(part 1 of 3)
# Autodesk Inventor assembly: Final
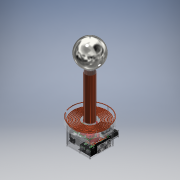
[picture p0: Inventor's stored thumbnail of the model, 180x180]
Saved by Autodesk Inventor 2019 (Build 230136000, 136)
## iProperties
Created: 2018-05-15
Part Number: Final
Document SubType Name: Assembly
Designer: Phil Erle
Author: Phil Erle
## Documents named in this file (78)
- C:\Users\Erle\Desktop\CAD\Final.iam
- C:\Users\Erle\Desktop\CAD\bottom.ipt
- C:\Users\Erle\Desktop\CAD\Elektronik_Gehäuse.ipt
- C:\Users\Erle\Desktop\CAD\Heatsink.ipt
- C:\Users\Erle\Desktop\CAD\EndStück_Caps.ipt
- C:\Users\Erle\Desktop\CAD\SeitenUntenVorne.ipt
- C:\Users\Erle\Desktop\CAD\SeitenUntenHinten.ipt
- C:\Users\Erle\Desktop\CAD\Cap.ipt
- C:\Users\Erle\Desktop\CAD\mid.ipt
- C:\Users\Erle\Desktop\CAD\MidStück_Caps.ipt
- C:\Users\Erle\Desktop\CAD\LogicHolder.ipt
- C:\Users\Erle\Desktop\CAD\NtHolder.ipt
- C:\Users\Erle\Desktop\CAD\SeitenUnten.ipt
- C:\Users\Erle\Desktop\CAD\ToslinkHalter.ipt
- C:\Users\Erle\Desktop\CAD\IGBT_Platine.ipt
- C:\Users\Erle\Desktop\CAD\GT175DA120U.ipt
- C:\Users\Erle\Desktop\CAD\Abstandshalter_12mm_M4.ipt
- C:\Users\Erle\Desktop\CAD\Normteile\Unterlegscheiben\din125-1-a_4_3-140_hv.ipt
- C:\Users\Erle\Desktop\CAD\CU6.ipt
- C:\Users\Erle\Desktop\CAD\CU5.ipt
- C:\Users\Erle\Desktop\CAD\Snubber.ipt
- C:\Users\Erle\Desktop\CAD\CU7.ipt
- C:\Users\Erle\Desktop\CAD\CU8.ipt
- C:\Users\Erle\Desktop\CAD\Normteile\Schrauben\M4\Zylinderkopf\din_en_iso_4762_m4x6.ipt
- C:\Users\Erle\Desktop\CAD\Normteile\Muttern\mutter_din934_m4-10.ipt
- C:\Users\Erle\Desktop\CAD\Cap_Platine.ipt
- C:\Users\Erle\Desktop\CAD\Main.ipt
- C:\Users\Erle\Desktop\CAD\SeitenOben.ipt
- C:\Users\Erle\Desktop\CAD\Abstandshalter_10mm.ipt
- C:\Users\Erle\Desktop\CAD\M5 Gewindestange.ipt
- C:\Users\Erle\Desktop\CAD\Normteile\Muttern\mutter_din934_m5-6.ipt
- C:\Users\Erle\Desktop\CAD\PlexiHalter1.ipt
- C:\Users\Erle\Desktop\CAD\PlexiHalter2.ipt
- C:\Users\Erle\Desktop\CAD\Primary.ipt
- C:\Users\Erle\Desktop\CAD\Seconday_End_Bottom.ipt
- C:\Users\Erle\Desktop\CAD\Seconday_End_Top.ipt
- C:\Users\Erle\Desktop\CAD\Normteile\Muttern\din1587-m5x0_8ricu3.ipt
- C:\Users\Erle\Desktop\CAD\Normteile\Muttern\mutter_din934_m6-6.ipt
- C:\Users\Erle\Desktop\CAD\Normteile\Muttern\din1587-m6x1ricu3.ipt
- C:\Users\Erle\Desktop\CAD\Secondary.ipt
- C:\Users\Erle\Desktop\CAD\Coil.ipt
- C:\Users\Erle\Desktop\CAD\M6 Gewindestange.ipt
- C:\Users\Erle\Desktop\CAD\TopLoad.ipt
- C:\Users\Erle\Desktop\CAD\primary_holder.ipt
- C:\Users\Erle\Desktop\CAD\Normteile\Schrauben\M3\din_en_iso_4762_m3x8.ipt
- C:\Users\Erle\Desktop\CAD\Normteile\Schrauben\M4\Zylinderkopf\din_en_iso_4762_m4x12.ipt
- C:\Users\Erle\Desktop\CAD\Normteile\Schrauben\M3\din_en_iso_4762_m3x10.ipt
- C:\Users\Erle\Desktop\CAD\Normteile\Muttern\mutter_din934_m3-6.ipt
- C:\Users\Erle\Desktop\CAD\Normteile\Schrauben\M3\din_en_iso_7991_m3x16.ipt
- C:\Users\Erle\Desktop\CAD\top.ipt
- C:\Users\Erle\Desktop\CAD\Strike_Rail.ipt
- C:\Users\Erle\Desktop\CAD\Power_Supply_S_90_18.ipt
- C:\Users\Erle\Desktop\CAD\M5 Gewindestange_Cap.ipt
- C:\Users\Erle\Desktop\CAD\Cu_Cap.ipt
- C:\Users\Erle\Desktop\CAD\Normteile\Unterlegscheiben\din125-1-a_5_3-140_hv.ipt
- C:\Users\Erle\Desktop\CAD\Platine_Gleichrichter.ipt
- C:\Users\Erle\Desktop\CAD\M6 Gewindestange_Unten.ipt
- C:\Users\Erle\Desktop\CAD\Gleichrichter.ipt
- C:\Users\Erle\Desktop\CAD\Netzfilter.ipt
- C:\Users\Erle\Desktop\CAD\Schalter.ipt
- C:\Users\Erle\Desktop\CAD\Netzstecker.ipt
- C:\Users\Erle\Desktop\CAD\Cap_CU_Oben.ipt
- C:\Users\Erle\Desktop\CAD\Normteile\Schrauben\M6\din_en_iso_4762_m6x10.ipt
- C:\Users\Erle\Desktop\CAD\Normteile\Schrauben\M5\din_en_iso_4762_m5x10.ipt
- C:\Users\Erle\Desktop\CAD\Normteile\Schrauben\M3\din_en_iso_4762_m3x25.ipt
- C:\Users\Erle\Desktop\CAD\Normteile\Schrauben\M3\din_en_iso_4762_m3x6.ipt
- C:\Users\Erle\Desktop\CAD\PrimaryCoil.ipt
- C:\Users\Erle\Desktop\CAD\Lüfter.ipt
- C:\Users\Erle\Desktop\CAD\Abstandshalter_5mm.ipt
- C:\Users\Erle\Desktop\CAD\GDT.ipt
- C:\Users\Erle\Desktop\CAD\Normteile\Schrauben\M3\din_en_iso_7991_m3x10.ipt
- C:\Users\Erle\Desktop\CAD\Normteile\Schrauben\M4\Zylinderkopf\din_en_iso_7991_m4x35.ipt
- C:\Users\Erle\Desktop\CAD\Rändelmutter.ipt
- C:\Users\Erle\Desktop\CAD\Lüftergitter.ipt
- C:\Users\Erle\Desktop\CAD\Normteile\Schrauben\M4\Zylinderkopf\din_en_iso_4762_m4x16.ipt
- C:\Users\Erle\Desktop\CAD\Normteile\Unterlegscheiben\din125-1-a_3_2-140_hv.ipt
- C:\Users\Erle\Desktop\CAD\CT.ipt
- C:\Users\Erle\Desktop\CAD\CT_Holder.ipt
## Components (478 placed, 77 different names)
1. bottom:1 — Flush:1, Flush:2, Mate:1, Mate:2, Mate:3, Mate:4, Mate:8, Mate:9, Mate:10, Mate:27, Mate:28, Mate:29, Mate:33, Mate:36, Mate:37, Mate:38, Mate:39, Mate:40, Mate:41, Mate:273, Mate:274, Mate:275, Flush:9, Flush:10, Flush:11, Flush:12, Mate:312, Mate:313, Mate:314, Mate:315, Mate:480, Mate:487, Mate:574, Mate:575, Mate:576, Mate:577, Mate:666, Mate:667, Mate:668, Mate:669, Mate:670, Mate:671, Mate:672, Mate:673, Mate:917, Mate:934, Mate:1121, Mate:1127, Mate:1132, Mate:1135
2. Elektronik_Gehäuse:1 — Mate:31, Mate:32, Mate:1106
3. Heatsink:1 — Mate:8, Mate:9, Mate:10, Mate:45, Mate:46, Mate:47, Mate:48, Mate:49, Mate:50, Mate:51, Mate:52, Mate:53, Mate:54, Mate:55, Mate:56, Mate:565, Mate:566, Angle:6, Mate:658, Mate:661, Mate:664, Mate:665, Mate:887, Mate:888, Mate:889, Mate:890, Mate:891, Mate:892, Mate:893, Mate:894, Mate:895, Mate:896, Mate:897, Mate:898
4. EndStück_Caps:1 — Mate:18, Mate:19, Mate:20, Mate:22, Mate:499, Mate:500, Mate:501, Mate:502, Flush:476, Flush:477, Flush:478, Flush:479, Mate:503, Mate:504, Mate:505, Mate:506
5. EndStück_Caps:2 — Mate:11, Mate:12, Mate:13, Mate:16, Mate:17, Mate:507, Mate:508, Mate:509, Mate:510
6. SeitenUntenVorne:1 — Mate:42, Mate:43, Mate:273, Mate:274, Mate:275, Mate:570, Mate:571, Mate:572, Mate:573, Angle:3, Mate:801, Mate:804, Mate:805, Mate:989, Mate:991
7. SeitenUntenHinten:1 — Mate:2, Mate:3, Mate:4, Mate:11, Mate:12, Mate:13, Mate:14, Mate:15, Mate:24, Mate:25, Mate:26, Mate:586, Mate:587, Mate:588, Mate:589, Mate:590, Mate:591, Mate:674, Mate:675, Mate:676, Mate:923, Mate:924, Mate:925, Mate:926, Mate:943, Mate:946, Mate:949, Mate:953, Mate:1145, Mate:1146, Mate:1147, Mate:1148
8. Cap:1 — Mate:14, Mate:17, Mate:18, Mate:19, Mate:23, Mate:523, Mate:524, Angle:5
9. Cap:2 — Mate:15, Mate:16, Mate:20, Mate:21, Mate:519, Mate:521, Mate:1042
10. mid:1 — Mate:24, Mate:25, Mate:26, Mate:211, Mate:212, Mate:213, Mate:215, Mate:219, Mate:222, Mate:224, Mate:225, Mate:227, Mate:232, Mate:233, Mate:234, Mate:245, Mate:246, Mate:247, Mate:249, Mate:252, Mate:253, Mate:255, Mate:259, Mate:268, Mate:269, Mate:270, Mate:271, Mate:272, Mate:276, Mate:277, Mate:278, Mate:279, Mate:280, Mate:281, Mate:282, Mate:363, Mate:484, Mate:490, Mate:491, Mate:492, Mate:603, Mate:604, Mate:605, Mate:606, Mate:607, Mate:608, Mate:609, Mate:610, Mate:611, Mate:612, Mate:613, Mate:614, Mate:615, Mate:616, Mate:617, Mate:697, Mate:698, Mate:706, Mate:709, Mate:710, Mate:711, Mate:712, Mate:713, Mate:714, Mate:715, Mate:716, Mate:717, Mate:718, Mate:719, Mate:720, Mate:721, Mate:722, Mate:723, Mate:724, Mate:725, Mate:735, Mate:736, Mate:737, Mate:738, Mate:741, Mate:742, Mate:743, Mate:744, Mate:745, Mate:746, Mate:747, Mate:750, Mate:1012, Mate:1136, Angle:7
11. MidStück_Caps:1 — Mate:21, Mate:22, Mate:23
12. LogicHolder:1 — Mate:27, Mate:28, Mate:29, Mate:31, Mate:32, Mate:485, Mate:486, Mate:917, Mate:932, Mate:933, Flush:484, Flush:485, Mate:1103, Mate:1105
13. NtHolder:1 — Mate:33, Mate:478, Mate:479, Mate:934, Mate:936, Mate:937, Mate:938, Mate:939, Mate:940, Mate:941, Flush:486, Flush:487, Flush:488, Flush:489, Mate:1086, Mate:1091, Mate:1093, Mate:1095
14. SeitenUnten:1 — Mate:37, Mate:38, Mate:41, Mate:846, Mate:847, Mate:848, Mate:849, Mate:854, Mate:855, Flush:490, Flush:491, Flush:971, Flush:492, Flush:493, Flush:494, Flush:495, Flush:496
15. SeitenUnten:2 — Mate:36, Mate:39, Mate:40, Mate:844, Mate:845, Mate:850, Mate:851, Mate:852, Mate:853, Flush:972, Flush:973, Flush:974, Flush:975, Flush:976, Flush:993, Flush:994, Flush:995
16. ToslinkHalter:1 — Mate:42, Mate:43, Mate:781, Mate:782, Mate:783, Mate:784, Mate:786, Mate:790
17. IGBT_Platine:1 — Mate:60, Mate:63, Mate:64, Mate:69, Mate:70, Mate:71, Mate:72, Mate:73, Mate:74, Mate:75, Mate:76
18. IGBT_Platine:2 — Mate:59, Mate:61, Mate:62, Mate:83, Mate:84, Mate:85, Mate:86
19. IGBT_Platine:3 — Mate:57, Mate:65, Mate:66, Mate:87, Mate:92, Mate:93, Mate:94, Mate:96, Mate:97, Mate:98
20. IGBT_Platine:4 — Mate:58, Mate:67, Mate:68, Mate:88, Mate:89, Mate:90, Mate:91
21. GT175DA120U:1 — Mate:48, Mate:49, Mate:50, Mate:57, Mate:65, Mate:66, Mate:95, Mate:119, Mate:120, Mate:121, Mate:705, Mate:731, Mate:733, Mate:734
22. GT175DA120U:2 — Mate:45, Mate:51, Mate:52, Mate:58, Mate:67, Mate:68, Mate:103, Mate:104, Mate:105, Mate:106, Mate:122, Mate:123, Mate:124, Mate:699, Mate:702, Mate:730, Mate:732
23. GT175DA120U:3 — Mate:47, Mate:55, Mate:56, Mate:59, Mate:61, Mate:62, Mate:99, Mate:100, Mate:101, Mate:102, Mate:116, Mate:117, Mate:118, Mate:703, Mate:704, Mate:726, Mate:728
24. GT175DA120U:4 — Mate:46, Mate:53, Mate:54, Mate:60, Mate:63, Mate:64, Mate:80, Mate:81, Mate:82, Mate:700, Mate:701, Mate:727, Mate:729
25. Abstandshalter_12mm_M4:1 — Mate:78, Mate:82, Mate:135, Mate:136, Mate:165
26. Abstandshalter_12mm_M4:2 — Mate:107, Mate:124, Mate:137, Mate:156
27. Abstandshalter_12mm_M4:3 — Mate:79, Mate:81, Mate:128, Mate:166
28. Abstandshalter_12mm_M4:4 — Mate:108, Mate:123, Mate:144, Mate:154
29. Abstandshalter_12mm_M4:5 — Mate:110, Mate:121, Mate:142, Mate:143, Mate:153
30. Abstandshalter_12mm_M4:6 — Mate:109, Mate:122, Mate:155
31. Abstandshalter_12mm_M4:7 — Mate:111, Mate:119, Mate:125, Mate:127, Mate:152
32. Abstandshalter_12mm_M4:8 — Mate:114, Mate:117, Mate:167
33. Abstandshalter_12mm_M4:9 — Mate:77, Mate:80, Mate:130, Mate:170
34. Abstandshalter_12mm_M4:10 — Mate:115, Mate:118, Mate:168
35. Abstandshalter_12mm_M4:15 — Mate:112, Mate:120, Mate:126, Mate:157
36. Abstandshalter_12mm_M4:16 — Mate:113, Mate:116, Mate:129, Mate:169
37. din125-1-a_4_3-140_hv:1 — Mate:72, Mate:73, Mate:77
38. din125-1-a_4_3-140_hv:2 — Mate:85, Mate:102, Mate:542, Mate:545
39. din125-1-a_4_3-140_hv:3 — Mate:70, Mate:76, Mate:78
40. din125-1-a_4_3-140_hv:4 — Mate:71, Mate:75, Mate:541, Mate:546
41. din125-1-a_4_3-140_hv:5 — Mate:94, Mate:96, Mate:110
42. din125-1-a_4_3-140_hv:6 — Mate:84, Mate:100, Mate:114
43. din125-1-a_4_3-140_hv:7 — Mate:93, Mate:95, Mate:112
44. din125-1-a_4_3-140_hv:8 — Mate:91, Mate:103, Mate:107
45. din125-1-a_4_3-140_hv:9 — Mate:89, Mate:106, Mate:108
46. din125-1-a_4_3-140_hv:10 — Mate:90, Mate:104, Mate:539, Mate:540
47. din125-1-a_4_3-140_hv:11 — Mate:86, Mate:99, Mate:115
48. din125-1-a_4_3-140_hv:12 — Mate:69, Mate:74, Mate:79
49. din125-1-a_4_3-140_hv:13 — Mate:83, Mate:101, Mate:113
50. din125-1-a_4_3-140_hv:14 — Mate:92, Mate:97, Mate:111
51. din125-1-a_4_3-140_hv:15 — Mate:88, Mate:105, Mate:109
52. din125-1-a_4_3-140_hv:16 — Mate:87, Mate:98, Mate:543, Mate:544
53. CU6:1 — Mate:125, Mate:126, Mate:127, Mate:131, Mate:132, Mate:133, Mate:134, Mate:151, Mate:158, Mate:161, Mate:162, Mate:186, Mate:187, Mate:199, Mate:763, Mate:764, Mate:779
54. CU5:1 — Mate:128, Mate:129, Mate:130, Mate:160, Mate:163, Mate:164, Mate:171, Mate:172, Mate:183, Mate:184, Mate:192, Mate:198, Mate:681, Mate:708, Mate:1077
55. Snubber:1 — Mate:131, Mate:132, Mate:171, Mate:176, Mate:178
56. Snubber:2 — Mate:133, Mate:134, Mate:145, Mate:175, Mate:177
57. Snubber:3 — Mate:138, Mate:140, Mate:172, Mate:174, Mate:180
58. Snubber:4 — Mate:139, Mate:141, Mate:146, Mate:173, Mate:179
59. CU7:1 — Mate:135, Mate:136, Mate:137, Mate:138, Mate:139, Mate:140, Mate:141, Mate:150, Mate:159, Mate:181, Mate:182, Mate:188, Mate:189, Mate:762, Mate:765, Mate:777
60. CU8:1 — Mate:142, Mate:143, Mate:144, Mate:145, Mate:146, Mate:147, Mate:148, Mate:149, Mate:185, Mate:190, Mate:191, Mate:200, Mate:458, Mate:682, Mate:707, Mate:1078
61. din_en_iso_4762_m4x6:1 — Mate:157, Mate:158
62. din_en_iso_4762_m4x6:2 — Mate:149, Mate:153
63. din_en_iso_4762_m4x6:3 — Mate:161, Mate:167
64. din_en_iso_4762_m4x6:4 — Mate:148, Mate:155
65. din_en_iso_4762_m4x6:5 — Mate:150, Mate:156
66. din_en_iso_4762_m4x6:6 — Mate:147, Mate:154
67. din_en_iso_4762_m4x6:7 — Mate:159, Mate:165
68. din_en_iso_4762_m4x6:8 — Mate:151, Mate:152
69. din_en_iso_4762_m4x6:9 — Mate:160, Mate:166
70. din_en_iso_4762_m4x6:10 — Mate:162, Mate:168
71. din_en_iso_4762_m4x6:11 — Mate:163, Mate:169
72. din_en_iso_4762_m4x6:12 — Mate:164, Mate:170
73. din_en_iso_4762_m4x6:13 — Mate:176, Mate:183, Mate:193
74. din_en_iso_4762_m4x6:14 — Mate:175, Mate:201, Mate:458
75. din_en_iso_4762_m4x6:15 — Mate:174, Mate:181, Mate:194
76. din_en_iso_4762_m4x6:16 — Mate:173, Mate:182, Mate:195
77. din_en_iso_4762_m4x6:17 — Mate:178, Mate:186, Mate:203
78. din_en_iso_4762_m4x6:18 — Mate:177, Mate:187, Mate:197
79. din_en_iso_4762_m4x6:19 — Mate:180, Mate:184, Mate:202
80. din_en_iso_4762_m4x6:20 — Mate:179, Mate:185, Mate:196
81. mutter_din934_m4-10:1 — Mate:188, Mate:195
82. mutter_din934_m4-10:2 — Mate:189, Mate:194
83. mutter_din934_m4-10:3 — Mate:190, Mate:196
84. mutter_din934_m4-10:4 — Mate:191, Mate:197
85. mutter_din934_m4-10:5 — Mate:198, Mate:202
86. mutter_din934_m4-10:6 — Mate:192, Mate:193
87. mutter_din934_m4-10:7 — Mate:200, Mate:201
88. mutter_din934_m4-10:8 — Mate:199, Mate:203
89. Main:1 — Mate:283, Mate:284, Mate:285, Mate:286, Mate:287, Mate:288, Mate:289, Mate:290, Mate:291, Mate:304, Mate:305, Mate:306, Mate:307, Mate:328, Mate:476, Mate:477, Mate:1126, Mate:1131, Mate:1133, Mate:1134
90. SeitenOben:1 — Mate:270, Mate:279, Mate:282
91. SeitenOben:2 — Mate:271, Mate:277, Mate:280, Mate:285
92. SeitenOben:3 — Mate:268, Mate:269, Mate:276, Mate:284
93. SeitenOben:4 — Mate:272, Mate:278, Mate:281, Mate:283
94. Abstandshalter_10mm:2 — Mate:212, Mate:234, Mate:235, Mate:596
95. Abstandshalter_10mm:3 — Mate:211, Mate:232, Mate:242, Mate:598, Mate:605
96. Abstandshalter_10mm:4 — Mate:213, Mate:233, Mate:595
97. Abstandshalter_10mm:7 — Mate:245, Mate:246, Mate:261, Mate:599
98. Abstandshalter_10mm:8 — Mate:219, Mate:259, Mate:260, Mate:594
99. Abstandshalter_10mm:9 — Mate:224, Mate:247, Mate:600
100. Abstandshalter_10mm:11 — Mate:225, Mate:255, Mate:256, Mate:602, Mate:603
101. Abstandshalter_10mm:14 — Mate:252, Mate:253, Mate:601
102. Abstandshalter_10mm:17 — Mate:215, Mate:249, Mate:593
103. Abstandshalter_10mm:19 — Mate:222, Mate:227, Mate:597, Mate:604
104. M5 Gewindestange:1 — Mate:288, Flush:10, Mate:298, Mate:299, Mate:319, Mate:323, Mate:324, Mate:367, Mate:1124, Mate:1125
105. M5 Gewindestange:2 — Mate:286, Flush:11, Mate:300, Mate:301, Mate:317, Mate:320, Mate:326, Mate:1122, Mate:1128
106. M5 Gewindestange:3 — Mate:287, Flush:9, Mate:302, Mate:303, Mate:318, Mate:321, Mate:327, Mate:1120, Mate:1123
107. M5 Gewindestange:4 — Mate:289, Flush:12, Mate:296, Mate:297, Mate:316, Mate:322, Mate:325, Mate:366, Mate:1129, Mate:1130
108. mutter_din934_m5-6:1 — Mate:302, Mate:309
109. mutter_din934_m5-6:2 — Mate:301, Mate:311
110. mutter_din934_m5-6:3 — Mate:299, Mate:307
111. mutter_din934_m5-6:4 — Mate:300, Mate:304
112. mutter_din934_m5-6:5 — Mate:303, Mate:305
113. mutter_din934_m5-6:6 — Mate:298, Mate:308
114. mutter_din934_m5-6:7 — Mate:296, Mate:310
115. mutter_din934_m5-6:8 — Mate:297, Mate:306
116. PlexiHalter1:1 — Mate:292, Mate:293, Mate:330, Mate:332, Mate:333, Mate:334, Mate:335
117. PlexiHalter1:2 — Mate:338, Mate:339, Mate:340, Mate:342, Mate:343, Mate:345, Mate:346, Mate:406, Mate:411, Mate:412, Mate:413, Mate:425, Mate:426, Mate:427, Mate:428
118. PlexiHalter2:1 — Mate:340, Mate:345, Mate:346, Mate:347, Mate:348, Mate:414, Mate:415, Mate:416, Mate:417
119. PlexiHalter2:2 — Mate:333, Mate:334, Mate:335, Mate:336, Mate:337, Mate:1107, Mate:1108, Mate:1109, Mate:1110, Mate:1111, Mate:1112, Mate:1113, Mate:1114, Mate:1115, Mate:1116, Mate:1117, Mate:1118
120. Primary:1 — Mate:308, Mate:309, Mate:310, Mate:311, Mate:328, Mate:356, Mate:357, Mate:358, Mate:359, Mate:360, Mate:366, Mate:367, Mate:368, Mate:369, Mate:370, Mate:371, Mate:372, Mate:373, Mate:374, Mate:375, Mate:376, Mate:377, Mate:378, Mate:379, Mate:380, Mate:381, Mate:382, Mate:383, Mate:384, Mate:385, Mate:386, Mate:387, Mate:388, Mate:389, Mate:390, Mate:391, Mate:392
121. Seconday_End_Bottom:1 — Mate:290, Mate:291, Mate:292, Mate:293, Mate:329, Mate:330, Mate:331, Mate:350, Mate:352, Flush:996, Flush:997, Flush:998, Flush:999
122. Seconday_End_Top:1 — Mate:338, Mate:339, Mate:341, Mate:343, Mate:344, Mate:351, Mate:353, Mate:354, Mate:430, Flush:432, Flush:14, Flush:15, Flush:16
123. din1587-m5x0_8ricu3:1 — Mate:313, Mate:321
124. din1587-m5x0_8ricu3:2 — Mate:316, Mate:325
125. din1587-m5x0_8ricu3:3 — Mate:315, Mate:320
126. din1587-m5x0_8ricu3:4 — Mate:312, Mate:322
127. din1587-m5x0_8ricu3:5 — Mate:318, Mate:327
128. din1587-m5x0_8ricu3:6 — Mate:314, Mate:323
129. din1587-m5x0_8ricu3:8 — Mate:319, Mate:324
130. din1587-m5x0_8ricu3:9 — Mate:317, Mate:326
131. mutter_din934_m6-6:1 — Mate:329, Mate:331, Mate:332, Mate:563
132. mutter_din934_m6-6:2 — Mate:341, Mate:342, Mate:344
133. din1587-m6x1ricu3:1 — Mate:336, Mate:337, Mate:564
134. din1587-m6x1ricu3:2 — Mate:347, Mate:348, Mate:429
135. Secondary:1 — Mate:349, Flush:13, Mate:350, Mate:351, Mate:352, Mate:353, Mate:393, Mate:394, Mate:395, Mate:396, Mate:401, Mate:402, Mate:403, Mate:404, Mate:474, Mate:842
136. Coil:1 — Mate:349, Flush:13
137. M6 Gewindestange:1 — Mate:354, Mate:355, Mate:429, Mate:435
138. TopLoad:1 — Mate:355, Mate:430, Flush:437
139. primary_holder:1 — Mate:358, Mate:451, Mate:452, Mate:454, Mate:455, Flush:475, Mate:475
140. primary_holder:2 — Mate:359, Mate:466, Mate:467, Mate:468, Flush:472
141. primary_holder:3 — Mate:368, Flush:438, Mate:438, Mate:440, Mate:442, Mate:443
142. primary_holder:4 — Mate:360, Mate:456, Mate:459, Mate:460, Flush:473
143. primary_holder:5 — Mate:357, Mate:437, Mate:444, Mate:445, Mate:447, Mate:449
144. primary_holder:6 — Mate:356, Mate:462, Flush:474, Mate:472, Mate:473, Mate:843
145. din_en_iso_4762_m3x8:1 — Mate:363, Mate:484, Mate:493
146. top:1 — Mate:435, Flush:437
147. Strike_Rail:1 — Mate:474, Mate:475
148. Power_Supply_S_90_18:1 — Mate:936, Mate:937, Mate:1097
149. Abstandshalter_10mm:25 — Mate:491, Mate:493, Mate:496, Mate:498
150. Abstandshalter_10mm:28 — Mate:490, Mate:492, Mate:497
151. M5 Gewindestange_Cap:1 — Mate:499, Flush:476, Mate:513, Mate:516, Mate:1141
152. M5 Gewindestange_Cap:2 — Mate:500, Flush:478, Mate:512, Mate:517, Mate:1142
153. M5 Gewindestange_Cap:3 — Mate:501, Flush:477, Mate:514, Mate:515, Mate:1143
154. M5 Gewindestange_Cap:4 — Mate:502, Flush:479, Mate:511, Mate:518, Mate:1144
155. Platine_Gleichrichter:1 — Mate:533, Mate:535, Mate:536, Mate:759, Mate:760, Mate:769, Mate:772, Mate:1015
156. Platine_Gleichrichter:2 — Mate:534, Mate:537, Mate:538, Mate:767, Mate:768, Mate:773, Mate:774
157. M6 Gewindestange_Unten:1 — Mate:563, Mate:564
158. CT:1 — Mate:1137, Flush:1001
159. CT:2 — Mate:1138, Flush:1000
160. CT_Holder:1 — Mate:1136, Mate:1137, Mate:1138, Flush:1000, Flush:1001, Mate:1139, Mate:1140, Angle:7
161. mutter_din934_m5-6:21 — Mate:1141, Mate:1147
162. mutter_din934_m5-6:22 — Mate:1142, Mate:1148
163. mutter_din934_m5-6:23 — Mate:1144, Mate:1145
164. mutter_din934_m5-6:24 — Mate:1143, Mate:1146
165. Lüftergitter:1 — Mate:1062, Mate:1063, Mate:1065, Mate:1070, Mate:1071, Mate:1072, Mate:1074
166. Lüftergitter:2 — Mate:1061, Mate:1064, Mate:1066, Mate:1067, Mate:1068, Mate:1069, Mate:1073
167. Lüftergitter:3 — Mate:1048, Mate:1053, Mate:1054, Mate:1055, Mate:1056, Mate:1057, Mate:1058
168. Lüftergitter:4 — Mate:1047, Mate:1049, Mate:1050, Mate:1051, Mate:1052, Mate:1059, Mate:1060
169. Cap_Platine:1 — Mate:242, Mate:597, Mate:598, Mate:625, Mate:629, Mate:641, Mate:642, Mate:644, Mate:655, Mate:685, Mate:692, Mate:813, Mate:817, Mate:818, Mate:829, Mate:830, Mate:833
170. Cap_Platine:2 — Mate:235, Mate:595, Mate:596, Mate:632, Mate:651, Mate:654, Mate:656, Mate:657, Mate:679, Mate:684, Mate:687, Mate:812, Mate:815, Mate:816, Mate:827, Mate:828, Mate:835
171. Cap_Platine:3 — Mate:261, Mate:599, Mate:600, Mate:618, Mate:619, Mate:636, Mate:637, Mate:646, Mate:648, Mate:755, Mate:823, Mate:825, Mate:826, Mate:837, Mate:840, Mate:841
172. Cap_Platine:4 — Mate:260, Mate:593, Mate:594, Mate:621, Mate:622, Mate:626, Mate:627, Mate:638, Mate:640, Mate:645, Mate:647, Mate:686, Mate:691, Mate:814, Mate:819, Mate:820, Mate:834, Mate:838, Mate:839
173. Cap_Platine:5 — Mate:256, Mate:601, Mate:602, Mate:623, Mate:624, Mate:630, Mate:631, Mate:649, Mate:650, Mate:652, Mate:653, Mate:680, Mate:683, Mate:806, Mate:807, Mate:808, Mate:809, Mate:810, Mate:811
174. Cap_Platine:6 — Mate:496, Mate:497, Mate:498, Mate:620, Mate:628, Mate:633, Mate:634, Mate:635, Mate:643, Mate:821, Mate:822, Mate:824, Mate:831, Mate:832, Mate:836
175. Netzstecker:1 — Mate:586, Mate:589, Mate:590, Mate:927, Mate:928, Flush:480, Flush:481
176. Netzstecker:2 — Mate:587, Mate:588, Mate:591, Mate:929, Mate:930, Flush:482, Flush:483
177. Abstandshalter_10mm:29 — Mate:608, Mate:616
178. Abstandshalter_10mm:30 — Mate:607, Mate:613
179. Abstandshalter_10mm:31 — Mate:609, Mate:615
180. Abstandshalter_10mm:32 — Mate:610, Mate:617
181. Abstandshalter_10mm:33 — Mate:606, Mate:614
182. Abstandshalter_10mm:34 — Mate:611, Mate:612
183. Schalter:1 — Mate:570, Mate:572, Angle:3, Angle:4, Mate:988
184. Schalter:2 — Mate:571, Mate:573, Angle:4, Mate:990
185. Netzfilter:1 — Mate:674, Mate:675, Mate:676, Mate:947, Mate:952
186. Gleichrichter:1 — Mate:565, Mate:566, Angle:6, Mate:1079, Mate:1080
187. Lüfter:1 — Mate:847, Mate:849, Mate:855, Mate:955, Mate:956, Mate:960, Mate:961, Mate:1048
188. Lüfter:2 — Mate:846, Mate:848, Mate:854, Mate:954, Mate:957, Mate:958, Mate:959, Mate:1047
189. Lüfter:3 — Mate:845, Mate:850, Mate:852, Mate:966, Mate:967, Mate:968, Mate:969, Mate:1062
190. Lüfter:4 — Mate:844, Mate:851, Mate:853, Mate:962, Mate:963, Mate:964, Mate:965, Mate:1061
191. Abstandshalter_5mm:1 — Mate:890, Mate:895, Mate:900
192. Abstandshalter_5mm:2 — Mate:888, Mate:893, Mate:899, Mate:903
193. Abstandshalter_5mm:3 — Mate:889, Mate:894, Mate:902
194. Abstandshalter_5mm:4 — Mate:892, Mate:898, Mate:901
195. Abstandshalter_5mm:5 — Mate:887, Mate:896
196. Abstandshalter_5mm:6 — Mate:891, Mate:897, Mate:904
197. GDT:1 — Mate:900, Mate:901, Mate:902, Mate:908, Mate:909, Mate:910, Mate:911, Mate:912, Mate:913
198. GDT:2 — Mate:899, Mate:903, Mate:904, Mate:905, Mate:906, Mate:907, Mate:914, Mate:915, Mate:916
199. Rändelmutter:1 — Mate:988, Mate:989
200. Rändelmutter:2 — Mate:990, Mate:991
201. PrimaryCoil:1 — Mate:842, Mate:843
202. Cu_Cap:1 — Mate:519, Mate:523, Mate:526, Mate:528, Mate:530, Mate:531, Mate:766, Mate:1017, Mate:1029, Mate:1031, Mate:1045
203. Cu_Cap:2 — Mate:521, Mate:524, Mate:525, Mate:527, Mate:529, Mate:532, Mate:761, Mate:1016, Mate:1027, Mate:1033, Mate:1046
204. Cap_CU_Oben:5 — Mate:630, Mate:631, Mate:632, Mate:688, Mate:689
205. Cap_CU_Oben:1 — Mate:621, Mate:627, Mate:629, Mate:694, Mate:695
206. Cap_CU_Oben:2 — Mate:618, Mate:619, Mate:620, Mate:756, Mate:757
207. Cap_CU_Oben:3 — Mate:622, Mate:626, Mate:628, Mate:696, Mate:758
208. Cap_CU_Oben:4 — Mate:623, Mate:624, Mate:625, Mate:690, Mate:693
209. din125-1-a_3_2-140_hv:1 — Mate:1087, Mate:1093, Mate:1094
210. din125-1-a_3_2-140_hv:5 — Mate:1100, Mate:1104, Mate:1106
211. din125-1-a_3_2-140_hv:6 — Mate:1101, Mate:1104, Mate:1105
212. din125-1-a_3_2-140_hv:7 — Mate:1099, Mate:1102
213. din125-1-a_3_2-140_hv:8 — Mate:1098, Mate:1102, Mate:1103
214. din125-1-a_3_2-140_hv:10 — Mate:1088, Mate:1094
215. din125-1-a_3_2-140_hv:11 — Mate:1089, Mate:1091, Mate:1092
216. din125-1-a_3_2-140_hv:12 — Mate:1090, Mate:1092
217. din125-1-a_3_2-140_hv:13 — Mate:1081, Mate:1085
218. din125-1-a_3_2-140_hv:14 — Mate:1083, Mate:1095, Mate:1096
219. din125-1-a_3_2-140_hv:15 — Mate:1082, Mate:1085, Mate:1086
220. din125-1-a_3_2-140_hv:16 — Mate:1084, Mate:1096, Mate:1097
221. din125-1-a_5_3-140_hv:1 — Mate:526, Mate:530, Mate:535, Mate:1015
222. din125-1-a_5_3-140_hv:2 — Mate:527, Mate:532, Mate:534, Mate:537
223. din125-1-a_5_3-140_hv:3 — Mate:528, Mate:531, Mate:538
224. din125-1-a_5_3-140_hv:4 — Mate:525, Mate:529, Mate:533, Mate:536
225. din125-1-a_5_3-140_hv:5 — Mate:1021, Mate:1026, Mate:1036
226. din125-1-a_5_3-140_hv:6 — Mate:1018, Mate:1028, Mate:1037
227. din125-1-a_5_3-140_hv:7 — Mate:1020, Mate:1028, Mate:1029
228. din125-1-a_5_3-140_hv:8 — Mate:1022, Mate:1030, Mate:1031
229. din125-1-a_5_3-140_hv:9 — Mate:1023, Mate:1030, Mate:1041
230. din125-1-a_5_3-140_hv:10 — Mate:1024, Mate:1032, Mate:1040
231. din125-1-a_5_3-140_hv:11 — Mate:1019, Mate:1026, Mate:1027
232. din125-1-a_5_3-140_hv:12 — Mate:1025, Mate:1032, Mate:1033
233. din125-1-a_5_3-140_hv:13 — Mate:1038, Mate:1041
234. din125-1-a_5_3-140_hv:14 — Mate:1034, Mate:1036
235. din125-1-a_5_3-140_hv:15 — Mate:1039, Mate:1040
236. din125-1-a_5_3-140_hv:16 — Mate:1035, Mate:1037, Mate:1042
237. din_en_iso_4762_m3x10:1 — Mate:393, Mate:405, Mate:407
238. din_en_iso_4762_m3x10:2 — Mate:394, Mate:410, Mate:422
239. din_en_iso_4762_m3x10:3 — Mate:396, Mate:409, Mate:423
240. din_en_iso_4762_m3x10:4 — Mate:395, Mate:408, Mate:424
241. din_en_iso_4762_m3x10:5 — Mate:401
242. din_en_iso_4762_m3x10:6 — Mate:402
243. din_en_iso_4762_m3x10:7 — Mate:404
244. din_en_iso_4762_m3x10:8 — Mate:403
245. din_en_iso_4762_m3x10:9 — Mate:666, Mate:667
246. din_en_iso_4762_m3x10:10 — Mate:668, Mate:671
247. din_en_iso_4762_m3x10:11 — Mate:670, Mate:673
248. din_en_iso_4762_m3x10:12 — Mate:669, Mate:672
249. din_en_iso_4762_m6x10:1 — Mate:684, Mate:688
250. din_en_iso_4762_m6x10:2 — Mate:682, Mate:707, Mate:1076
251. din_en_iso_4762_m3x8:2 — Mate:698, Mate:720
252. din_en_iso_4762_m3x8:3 — Mate:712, Mate:750
253. din_en_iso_4762_m3x8:4 — Mate:713, Mate:717
254. din_en_iso_4762_m3x8:5 — Mate:699, Mate:702
255. din_en_iso_4762_m3x8:6 — Mate:709, Mate:721
256. din_en_iso_4762_m3x8:7 — Mate:715, Mate:716
257. din_en_iso_4762_m3x8:8 — Mate:700, Mate:701
258. din_en_iso_4762_m3x8:9 — Mate:703, Mate:704
259. din_en_iso_4762_m3x8:10 — Mate:714, Mate:718
260. din_en_iso_4762_m3x8:11 — Mate:697, Mate:741
261. din_en_iso_4762_m3x8:12 — Mate:711, Mate:723
262. din_en_iso_4762_m3x8:13 — Mate:710, Mate:722
263. din_en_iso_4762_m3x8:14 — Mate:705, Mate:733
264. din_en_iso_4762_m3x8:15 — Mate:706, Mate:719
265. din_en_iso_4762_m3x8:16 — Mate:726, Mate:728
266. din_en_iso_4762_m3x8:17 — Mate:736, Mate:745
267. din_en_iso_4762_m3x8:18 — Mate:727, Mate:729
268. din_en_iso_4762_m3x8:19 — Mate:724, Mate:742
269. din_en_iso_4762_m3x8:21 — Mate:737, Mate:744
270. din_en_iso_4762_m3x8:22 — Mate:738, Mate:743
271. din_en_iso_4762_m3x10:18 — Mate:1011, Mate:1139, Mate:1140
272. din_en_iso_4762_m3x8:24 — Mate:731, Mate:734
273. din_en_iso_4762_m3x8:25 — Mate:730, Mate:732
274. din_en_iso_4762_m3x8:26 — Mate:735, Mate:747
275. din_en_iso_4762_m3x8:27 — Mate:725, Mate:746
276. din_en_iso_4762_m3x25:1 — Mate:781, Mate:784, Mate:789, Mate:794, Mate:795, Mate:796, Mate:803
277. din_en_iso_4762_m3x25:2 — Mate:782, Mate:783, Mate:785, Mate:787, Mate:788, Mate:793, Mate:802
278. din_en_iso_4762_m3x6:1 — Mate:808, Mate:811
279. din_en_iso_4762_m3x6:2 — Mate:822, Mate:832
280. din_en_iso_4762_m3x6:3 — Mate:821, Mate:831
281. din_en_iso_4762_m3x6:4 — Mate:820, Mate:839
282. din_en_iso_4762_m3x6:5 — Mate:825, Mate:841
283. din_en_iso_4762_m3x6:6 — Mate:807, Mate:809
284. din_en_iso_4762_m3x6:7 — Mate:818, Mate:830
285. din_en_iso_4762_m3x6:8 — Mate:826, Mate:840
286. din_en_iso_4762_m3x6:9 — Mate:806, Mate:810
287. din_en_iso_4762_m3x6:10 — Mate:812, Mate:827
288. din_en_iso_4762_m3x6:11 — Mate:824, Mate:836
289. din_en_iso_4762_m3x6:12 — Mate:819, Mate:838
290. din_en_iso_4762_m3x6:13 — Mate:823, Mate:837
291. din_en_iso_4762_m3x6:14 — Mate:817, Mate:829
292. din_en_iso_4762_m3x6:15 — Mate:816, Mate:828
293. din_en_iso_4762_m3x6:16 — Mate:814, Mate:834
294. din_en_iso_4762_m3x6:17 — Mate:815, Mate:835
295. din_en_iso_4762_m3x6:18 — Mate:813, Mate:833
296. din_en_iso_4762_m3x6:19 — Mate:909, Mate:911
297. din_en_iso_4762_m3x6:20 — Mate:906, Mate:916
298. din_en_iso_4762_m3x6:21 — Mate:905, Mate:915
299. din_en_iso_4762_m3x6:22 — Mate:910, Mate:912
300. din_en_iso_4762_m3x6:23 — Mate:907, Mate:914
301. din_en_iso_4762_m3x6:24 — Mate:908, Mate:913
302. din_en_iso_4762_m3x10:15 — Mate:924, Mate:926, Mate:944
303. din_en_iso_4762_m3x10:16 — Mate:923, Mate:925, Mate:951
304. din_en_iso_4762_m4x12:1 — Mate:369, Mate:374, Mate:471
305. din_en_iso_4762_m4x12:2 — Mate:371, Mate:373, Mate:465
306. din_en_iso_4762_m4x12:3 — Mate:372, Mate:376, Mate:464
307. din_en_iso_4762_m4x12:4 — Mate:370, Mate:375, Mate:463
308. din_en_iso_4762_m4x12:5 — Mate:384, Mate:389, Mate:448
309. din_en_iso_4762_m4x12:6 — Mate:383, Mate:391, Mate:461
310. din_en_iso_4762_m4x12:7 — Mate:380, Mate:390, Mate:457
311. din_en_iso_4762_m4x12:8 — Mate:382, Mate:386, Mate:450
312. din_en_iso_4762_m4x12:9 — Mate:379, Mate:387, Mate:453
313. din_en_iso_4762_m4x12:10 — Mate:381, Mate:385, Mate:439
314. din_en_iso_4762_m4x12:11 — Mate:378, Mate:392, Mate:441
315. din_en_iso_4762_m4x12:12 — Mate:377, Mate:388, Mate:446
316. din_en_iso_4762_m4x6:21 — Mate:543, Mate:544
317. din_en_iso_4762_m4x6:22 — Mate:539, Mate:540
318. din_en_iso_4762_m4x6:23 — Mate:541, Mate:546
319. din_en_iso_4762_m4x6:24 — Mate:542, Mate:545
320. din_en_iso_4762_m4x12:13 — Mate:574, Mate:576
321. din_en_iso_4762_m4x12:14 — Mate:575, Mate:577
322. din_en_iso_4762_m4x16:1 — Mate:1079, Mate:1080
323. din_en_iso_4762_m5x10:1 — Mate:762, Mate:765, Mate:778
324. din_en_iso_4762_m5x10:2 — Mate:760, Mate:769, Mate:1018, Mate:1020, Mate:1035
325. din_en_iso_4762_m5x10:3 — Mate:761, Mate:1016, Mate:1044
326. din_en_iso_4762_m5x10:4 — Mate:759, Mate:772, Mate:1019, Mate:1021, Mate:1034
327. din_en_iso_4762_m5x10:5 — Mate:768, Mate:774, Mate:1022, Mate:1023, Mate:1038
328. din_en_iso_4762_m5x10:6 — Mate:763, Mate:764, Mate:780
329. din_en_iso_4762_m5x10:7 — Mate:766, Mate:1017, Mate:1043
330. din_en_iso_4762_m5x10:8 — Mate:767, Mate:773, Mate:1024, Mate:1025, Mate:1039
331. din_en_iso_4762_m6x10:3 — Mate:680, Mate:689
332. din_en_iso_4762_m6x10:4 — Mate:681, Mate:708, Mate:1075
333. din_en_iso_4762_m6x10:5 — Mate:685, Mate:693
334. din_en_iso_4762_m6x10:6 — Mate:692, Mate:694
335. din_en_iso_4762_m6x10:7 — Mate:691, Mate:696
336. din_en_iso_4762_m6x10:8 — Mate:686, Mate:695
337. din_en_iso_4762_m6x10:9 — Mate:683, Mate:690
338. din_en_iso_4762_m6x10:10 — Mate:679, Mate:687
339. din_en_iso_4762_m6x10:11 — Mate:753, Mate:758
340. din_en_iso_4762_m6x10:12 — Mate:754, Mate:757
341. din_en_iso_4762_m6x10:13 — Mate:751, Mate:755
342. din_en_iso_4762_m6x10:14 — Mate:752, Mate:756
343. din_en_iso_7991_m3x16:1 — Mate:425, Flush:16, Mate:431
344. din_en_iso_7991_m3x16:2 — Mate:427, Flush:432, Mate:432
345. din_en_iso_7991_m3x16:3 — Mate:426, Flush:14, Mate:434
346. din_en_iso_7991_m3x16:4 — Mate:428, Flush:15, Mate:433
347. din_en_iso_7991_m3x10:1 — Mate:930, Flush:482, Mate:942
348. din_en_iso_7991_m3x10:2 — Mate:928, Flush:480, Mate:948
349. din_en_iso_7991_m3x10:3 — Mate:929, Flush:483, Mate:945
350. din_en_iso_7991_m3x10:4 — Mate:927, Flush:481, Mate:950
351. din_en_iso_7991_m3x10:5 — Mate:932, Flush:484, Mate:1100, Mate:1101
352. din_en_iso_7991_m3x10:6 — Mate:933, Flush:485, Mate:1098, Mate:1099
353. din_en_iso_7991_m3x10:7 — Mate:939, Flush:489, Mate:1081, Mate:1082
354. din_en_iso_7991_m3x10:8 — Mate:938, Flush:488, Mate:1089, Mate:1090
355. din_en_iso_7991_m3x10:9 — Mate:940, Flush:487, Mate:1083, Mate:1084
356. din_en_iso_7991_m3x10:10 — Mate:941, Flush:486, Mate:1087, Mate:1088
357. din_en_iso_7991_m3x16:5 — Mate:1116, Flush:997
358. din_en_iso_7991_m3x16:6 — Mate:1118, Flush:996
359. din_en_iso_7991_m3x16:7 — Mate:1117, Flush:998
360. din_en_iso_7991_m3x16:8 — Mate:1115, Flush:999
361. din_en_iso_7991_m4x35:1 — Mate:962, Flush:974, Mate:994, Mate:1064
362. din_en_iso_7991_m4x35:2 — Mate:963, Flush:976, Mate:997, Mate:1066
363. din_en_iso_7991_m4x35:3 — Mate:964, Flush:995, Mate:1002
364. din_en_iso_7991_m4x35:4 — Mate:965, Flush:994, Mate:1004
365. din_en_iso_7991_m4x35:5 — Mate:966, Flush:993, Mate:1001
366. din_en_iso_7991_m4x35:6 — Mate:967, Flush:975, Mate:1000
367. din_en_iso_7991_m4x35:7 — Mate:968, Flush:972, Mate:992, Mate:1063
368. din_en_iso_7991_m4x35:8 — Mate:969, Flush:973, Mate:996, Mate:1065
369. din_en_iso_7991_m4x35:9 — Mate:955, Flush:490, Mate:971
370. din_en_iso_7991_m4x35:10 — Mate:956, Flush:491, Mate:972, Mate:1053
371. din_en_iso_7991_m4x35:11 — Mate:957, Flush:971, Mate:986
372. din_en_iso_7991_m4x35:12 — Mate:958, Flush:493, Mate:974
373. din_en_iso_7991_m4x35:13 — Mate:959, Flush:494, Mate:975, Mate:1050
374. din_en_iso_7991_m4x35:14 — Mate:960, Flush:496, Mate:977, Mate:1054
375. din_en_iso_7991_m4x35:15 — Mate:961, Flush:492, Mate:973
376. din_en_iso_7991_m4x35:16 — Mate:954, Flush:495, Mate:976, Mate:1049
377. mutter_din934_m3-6:1 — Mate:409, Mate:413, Mate:423
378. mutter_din934_m3-6:2 — Mate:408, Mate:412, Mate:424
379. mutter_din934_m3-6:3 — Mate:410, Mate:411, Mate:422
380. mutter_din934_m3-6:4 — Mate:405, Mate:406, Mate:407
381. mutter_din934_m3-6:5 — Mate:417, Mate:432
382. mutter_din934_m3-6:6 — Mate:416, Mate:431
383. mutter_din934_m3-6:7 — Mate:414, Mate:433
384. mutter_din934_m3-6:8 — Mate:415, Mate:434
385. mutter_din934_m3-6:33
386. mutter_din934_m3-6:31
387. mutter_din934_m3-6:34
388. mutter_din934_m3-6:32
389. mutter_din934_m3-6:9 — Mate:661
390. mutter_din934_m3-6:10 — Mate:658
391. mutter_din934_m3-6:11 — Mate:664
392. mutter_din934_m3-6:12 — Mate:665
393. mutter_din934_m3-6:13 — Mate:788, Mate:792, Mate:800
394. mutter_din934_m3-6:14 — Mate:793, Mate:800, Mate:801
395. mutter_din934_m3-6:15 — Mate:796, Mate:799
396. mutter_din934_m3-6:16 — Mate:795, Mate:797, Mate:798
397. mutter_din934_m3-6:17 — Mate:787, Mate:791, Mate:792
398. mutter_din934_m3-6:18 — Mate:794, Mate:798, Mate:799
399. mutter_din934_m3-6:19 — Mate:785, Mate:786, Mate:791
400. mutter_din934_m3-6:20 — Mate:789, Mate:790, Mate:797
401. mutter_din934_m3-6:21 — Mate:803, Mate:804
402. mutter_din934_m3-6:22 — Mate:802, Mate:805
403. mutter_din934_m3-6:23 — Mate:951, Mate:952
404. mutter_din934_m3-6:24 — Mate:948, Mate:949
405. mutter_din934_m3-6:25 — Mate:942, Mate:943
406. mutter_din934_m3-6:26 — Mate:945, Mate:946
407. mutter_din934_m3-6:27 — Mate:944, Mate:947
408. mutter_din934_m3-6:28 — Mate:950, Mate:953
409. mutter_din934_m3-6:30 — Mate:1011, Mate:1012
410. mutter_din934_m3-6:35 — Mate:1107, Mate:1111
411. mutter_din934_m3-6:36 — Mate:1108, Mate:1112
412. mutter_din934_m3-6:37 — Mate:1109, Mate:1110
413. mutter_din934_m3-6:38 — Mate:1113, Mate:1114
414. mutter_din934_m4-10:21 — Mate:478, Mate:479, Mate:480
415. mutter_din934_m4-10:22 — Mate:485, Mate:486, Mate:487
416. mutter_din934_m4-10:9 — Mate:440, Mate:441, Mate:442
417. mutter_din934_m4-10:10 — Mate:438, Mate:439, Mate:443
418. mutter_din934_m4-10:11 — Mate:445, Mate:446, Mate:447
419. mutter_din934_m4-10:12 — Mate:444, Mate:448, Mate:449
420. mutter_din934_m4-10:13 — Mate:450, Mate:451, Mate:455
421. mutter_din934_m4-10:14 — Mate:452, Mate:453, Mate:454
422. mutter_din934_m4-10:15 — Mate:471, Mate:472, Mate:473
423. mutter_din934_m4-10:16 — Mate:456, Mate:457, Mate:459
424. mutter_din934_m4-10:17 — Mate:464, Mate:467, Mate:468
425. mutter_din934_m4-10:18 — Mate:465, Mate:466
426. mutter_din934_m4-10:19 — Mate:460, Mate:461
427. mutter_din934_m4-10:20 — Mate:462, Mate:463
428. mutter_din934_m4-10:27 — Mate:972, Mate:1056
429. mutter_din934_m4-10:28 — Mate:975, Mate:1052
430. mutter_din934_m4-10:29 — Mate:974, Mate:1060
431. mutter_din934_m4-10:30 — Mate:973, Mate:1058
432. mutter_din934_m4-10:31 — Mate:986, Mate:1059
433. mutter_din934_m4-10:32 — Mate:976, Mate:1051
434. mutter_din934_m4-10:33 — Mate:971, Mate:1055
435. mutter_din934_m4-10:34 — Mate:977, Mate:1057
436. mutter_din934_m4-10:35 — Mate:1004, Mate:1069
437. mutter_din934_m4-10:36 — Mate:997, Mate:1067
438. mutter_din934_m4-10:37 — Mate:996, Mate:1074
439. mutter_din934_m4-10:38 — Mate:994, Mate:1073
440. mutter_din934_m4-10:39 — Mate:1001, Mate:1071
441. mutter_din934_m4-10:40 — Mate:1002, Mate:1068
442. mutter_din934_m4-10:41 — Mate:992, Mate:1072
443. mutter_din934_m4-10:42 — Mate:1000, Mate:1070
444. mutter_din934_m5-6:13 — Mate:1123, Mate:1126
445. mutter_din934_m5-6:15 — Mate:1129, Mate:1132
446. mutter_din934_m5-6:16 — Mate:1130, Mate:1133
447. mutter_din934_m5-6:17 — Mate:1128, Mate:1131
448. mutter_din934_m5-6:18 — Mate:1122, Mate:1127
449. mutter_din934_m5-6:19 — Mate:1120, Mate:1121
450. mutter_din934_m5-6:20 — Mate:1125, Mate:1134
451. mutter_din934_m5-6:14 — Mate:1124, Mate:1135
452. mutter_din934_m5-6:9 — Mate:779, Mate:780
453. mutter_din934_m5-6:10 — Mate:777, Mate:778
454. mutter_din934_m5-6:11 — Mate:1043, Mate:1045
455. mutter_din934_m5-6:12 — Mate:1044, Mate:1046
456. mutter_din934_m6-6:3 — Mate:633, Mate:634, Mate:753
457. mutter_din934_m6-6:4 — Mate:640, Mate:647
458. mutter_din934_m6-6:5 — Mate:656, Mate:657
459. mutter_din934_m6-6:6 — Mate:641, Mate:655
460. mutter_din934_m6-6:7 — Mate:642, Mate:644
461. mutter_din934_m6-6:8 — Mate:636, Mate:646, Mate:752
462. mutter_din934_m6-6:9 — Mate:635, Mate:643, Mate:754
463. mutter_din934_m6-6:10 — Mate:649, Mate:652
464. mutter_din934_m6-6:11 — Mate:637, Mate:648, Mate:751
465. mutter_din934_m6-6:12 — Mate:651, Mate:654
466. mutter_din934_m6-6:13 — Mate:638, Mate:645
467. mutter_din934_m6-6:14 — Mate:650, Mate:653
468. mutter_din934_m6-6:17 — Mate:1076, Mate:1078
469. mutter_din934_m6-6:18 — Mate:1075, Mate:1077
470. din1587-m5x0_8ricu3:10 — Mate:510, Mate:518
471. din1587-m5x0_8ricu3:11 — Mate:507, Mate:516
472. din1587-m5x0_8ricu3:12 — Mate:509, Mate:515
473. din1587-m5x0_8ricu3:13 — Mate:508, Mate:517
474. din1587-m5x0_8ricu3:14 — Mate:503, Mate:514